# Autodesk Inventor assembly: cabeça_inferior
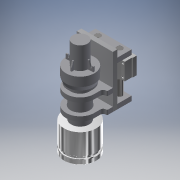
[picture p0: Inventor's stored thumbnail of the model, 180x180]
Saved by Autodesk Inventor 2018 (Build 220112000, 112)
## iProperties
Created: 2018-05-10
Part Number: cabeça_inferior
Material: Genérico
Document SubType Name: Assembly
Designer: Georgines
Mass: 1069.3 g
Surface Area: 1697.31 cm^2
Volume: 551.873 cm^3
Density: 1.93759 g/cm^3
Author: Georgines
## Documents named in this file (8)
- C:\Users\Georgines\Documents\EstacaoBGA\Peças 3D\cabeça_inferior.iam
- C:\Users\Georgines\Documents\EstacaoBGA\Peças 3D\bocal_de_aquecimento.ipt
- C:\Users\Georgines\Documents\EstacaoBGA\Peças 3D\soprador_original.ipt
- C:\Users\Georgines\Documents\EstacaoBGA\Peças 3D\suporte_boca_soprador.ipt
- C:\Users\Georgines\Documents\EstacaoBGA\Peças 3D\SCS12UU.iam
- C:\Users\Georgines\Documents\EstacaoBGA\Peças 3D\SuporteAquecedor.ipt
- C:\Users\Georgines\Documents\EstacaoBGA\Peças 3D\guia_linear_12mm_150mm.ipt
- C:\Users\Georgines\Documents\EstacaoBGA\Peças 3D\SuporteGuiasCabeçasAquecimento.ipt
## Components (11 placed, 7 different names)
1. bocal_de_aquecimento:1 — Inserir:1, Alinhamento:2
2. soprador_original:1 — Inserir:1, Coincidência:3
3. suporte_boca_soprador:1 — Alinhamento:2, Coincidência:1, Coincidência:2, Alinhamento:3, Alinhamento:4, Alinhamento:5, Coincidência:12, Alinhamento:9, Alinhamento:11
4. SCS12UU:1 [sub-assembly] — Coincidência:10, Alinhamento:7, Alinhamento:8, Coincidência:13
5. SCS12UU:2 [sub-assembly] — Coincidência:11, Alinhamento:7, Alinhamento:8
6. SuporteAquecedor:1 — Coincidência:2, Alinhamento:3
7. SuporteAquecedor:2 — Coincidência:1, Alinhamento:4, Coincidência:3, Alinhamento:5
8. guia_linear_12mm_150mm:1 — Coincidência:5, Coincidência:8, Coincidência:11, Alinhamento:12
9. guia_linear_12mm_150mm:2 — Coincidência:4, Coincidência:7, Coincidência:10, Alinhamento:13, Alinhamento:14
10. SuporteGuiasCabeçasAquecimento:1 — Coincidência:7, Coincidência:8, Coincidência:12, Alinhamento:9, Alinhamento:14
11. SuporteGuiasCabeçasAquecimento:2 — Coincidência:4, Coincidência:5, Coincidência:13, Alinhamento:11, Alinhamento:12, Alinhamento:13
## Relationships (23: Flush 11, Mate 11, Insert 1)
- Inserir:1 (-2.5 mm): bocal_de_aquecimento:1 ↔ soprador_original:1
- Alinhamento:2 [Flush]: bocal_de_aquecimento:1 ↔ suporte_boca_soprador:1
- Coincidência:1 [Mate]: suporte_boca_soprador:1 ↔ SuporteAquecedor:2
- Coincidência:2 [Mate]: suporte_boca_soprador:1 ↔ SuporteAquecedor:1
- Alinhamento:3 [Flush]: suporte_boca_soprador:1 ↔ SuporteAquecedor:1
- Alinhamento:4 [Flush]: suporte_boca_soprador:1 ↔ SuporteAquecedor:2
- Coincidência:3 [Mate]: soprador_original:1 ↔ SuporteAquecedor:2
- Alinhamento:5 [Flush]: suporte_boca_soprador:1 ↔ SuporteAquecedor:2
- Coincidência:4 [Mate]: guia_linear_12mm_150mm:2 ↔ SuporteGuiasCabeçasAquecimento:2
- Coincidência:5 [Mate]: guia_linear_12mm_150mm:1 ↔ SuporteGuiasCabeçasAquecimento:2
- Coincidência:7 [Mate]: guia_linear_12mm_150mm:2 ↔ SuporteGuiasCabeçasAquecimento:1
- Coincidência:8 [Mate]: guia_linear_12mm_150mm:1 ↔ SuporteGuiasCabeçasAquecimento:1
- Coincidência:10 [Mate]: SCS12UU:1 ↔ guia_linear_12mm_150mm:2
- Coincidência:11 [Mate]: SCS12UU:2 ↔ guia_linear_12mm_150mm:1
- Alinhamento:7 [Flush]: SCS12UU:1 ↔ SCS12UU:2
- Alinhamento:8 [Flush]: SCS12UU:1 ↔ SCS12UU:2
- Coincidência:12 [Mate]: suporte_boca_soprador:1 ↔ SuporteGuiasCabeçasAquecimento:1
- Alinhamento:9 [Flush]: suporte_boca_soprador:1 ↔ SuporteGuiasCabeçasAquecimento:1
- Coincidência:13 [Mate]: SCS12UU:1 ↔ SuporteGuiasCabeçasAquecimento:2
- Alinhamento:11 [Flush]: suporte_boca_soprador:1 ↔ SuporteGuiasCabeçasAquecimento:2
- Alinhamento:12 [Flush]: guia_linear_12mm_150mm:1 ↔ SuporteGuiasCabeçasAquecimento:2
- Alinhamento:13 [Flush]: guia_linear_12mm_150mm:2 ↔ SuporteGuiasCabeçasAquecimento:2
- Alinhamento:14 [Flush]: guia_linear_12mm_150mm:2 ↔ SuporteGuiasCabeçasAquecimento:1
